# Autodesk Inventor assembly: Robot_Rev1
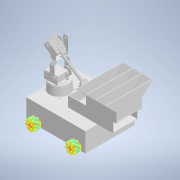
[picture p0: Inventor's stored thumbnail of the model, 180x180]
Saved by Autodesk Inventor 2020 (Build 240168000, 168)
## iProperties
Created: 2021-12-09
Part Number: Robot_Rev1
Document SubType Name: Assembly
Designer: danie
Author: danie
## Documents named in this file (8)
- C:\Users\danie\Documents\Capstone\Solidworks\Robot_Rev1.iam
- C:\Users\danie\Documents\Capstone\Solidworks\Lower Chassis.ipt
- C:\Users\danie\Documents\Capstone\Solidworks\UpperChassis_Base.ipt
- C:\Users\danie\Documents\Capstone\Solidworks\MECHANUM WHEEL.iam
- C:\Users\danie\Documents\Capstone\Solidworks\ShootingMech_Housing.ipt
- C:\Users\danie\Documents\Capstone\Solidworks\AL5D_2017_12_17.iam
- C:\Users\danie\Documents\Capstone\Solidworks\BeadCompartments_2.ipt
- C:\Users\danie\Documents\Capstone\Solidworks\False_Bottom.ipt
## Components (10 placed, 7 different names)
1. Lower Chassis:1 — Rigid:1
2. UpperChassis_Base:1 — Rigid:1
3. MECHANUM WHEEL:2 [sub-assembly]
4. MECHANUM WHEEL:3 [sub-assembly]
5. MECHANUM WHEEL:4 [sub-assembly]
6. MECHANUM WHEEL:5 [sub-assembly]
7. ShootingMech_Housing:1
8. AL5D_2017_12_17:1 [sub-assembly]
9. BeadCompartments_2:1
10. False_Bottom:1
## Relationships (1: WeldJoint 1)
- Rigid:1 [WeldJoint]: Lower Chassis:1 ↔ UpperChassis_Base:1
